# Autodesk Inventor assembly: withtraces
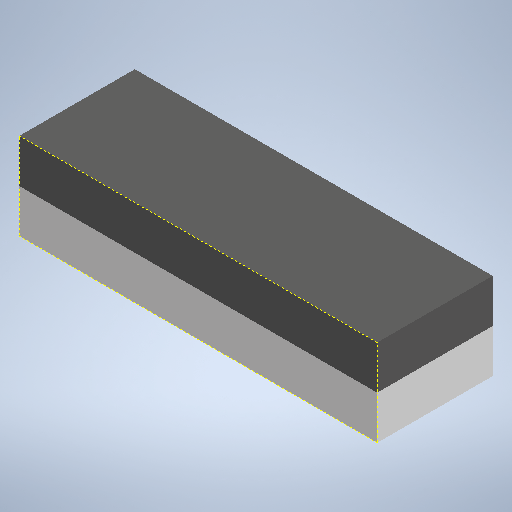
[picture p0: Inventor's stored thumbnail of the model, 512x512]
Saved by Autodesk Inventor 2025 (Build 290162000, 162)
## iProperties
Created: 2024-08-06
Part Number: withtraces
Document SubType Name: Assembly
Designer: ethan
Author: ethan
## Documents named in this file (2)
- C:\Users\ethan\Documents\GitHub\3D-Pants\Net_cards\chipcase\withtraces.iam
- C:\Users\ethan\Documents\GitHub\3D-Pants\Net_cards\chipcase\Bottom.ipt
## Components (2 placed, 1 different names)
1. Bottom:1 — Mate:1, Flush:1, Flush:2
2. Bottom:2 — Mate:1, Flush:1, Flush:2
## Relationships (3: Flush 2, Mate 1)
- Mate:1: Bottom:1 ↔ Bottom:2
- Flush:1: Bottom:1 ↔ Bottom:2
- Flush:2: Bottom:1 ↔ Bottom:2
